# Autodesk Inventor assembly: rotor-housing-assembly
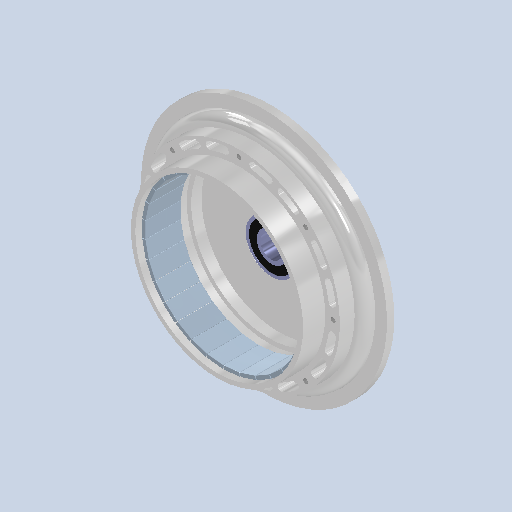
[picture p0: Inventor's stored thumbnail of the model, 512x512]
Saved by Autodesk Inventor 2022 (Build 260153000, 153)
## iProperties
Created: 2025-01-12
Part Number: rotor-housing-assembly
Document SubType Name: Assembly
Designer: Home
Author: Home
## Documents named in this file (4)
- D:\YandexDisk\Voltbro\xSets\components\HubWheel-10\rotor-housing-assembly.iam
- D:\YandexDisk\Voltbro\xSets\components\HubWheel-10\rotor-disc.ipt
- D:\YandexDisk\Voltbro\xSets\components\HubWheel-10\magnet_11x24-x2_5.ipt
- D:\YandexDisk\Voltbro\xSets\components\HubWheel-10\components\bearings\6202-2rs_15x35x11.ipt
## Components (32 placed, 3 different names)
1. rotor-disc:1 — Mate:4, Tangent:1, Tangent:2, Flush:1, Insert:1
2. 6202-2rs_15x35x11:1 — Insert:1
3. magnet_11x24-x2_5:1 — Mate:3, Tangent:1, Tangent:2, Flush:1
4. magnet_11x24-x2_5:2
5. magnet_11x24-x2_5:3
6. magnet_11x24-x2_5:4
7. magnet_11x24-x2_5:5
8. magnet_11x24-x2_5:6
9. magnet_11x24-x2_5:7
10. magnet_11x24-x2_5:8
11. magnet_11x24-x2_5:9
12. magnet_11x24-x2_5:10
13. magnet_11x24-x2_5:11
14. magnet_11x24-x2_5:12
15. magnet_11x24-x2_5:13
16. magnet_11x24-x2_5:14
17. magnet_11x24-x2_5:15
18. magnet_11x24-x2_5:16
19. magnet_11x24-x2_5:17
20. magnet_11x24-x2_5:18
21. magnet_11x24-x2_5:19
22. magnet_11x24-x2_5:20
23. magnet_11x24-x2_5:21
24. magnet_11x24-x2_5:22
25. magnet_11x24-x2_5:23
26. magnet_11x24-x2_5:24
27. magnet_11x24-x2_5:25
28. magnet_11x24-x2_5:26
29. magnet_11x24-x2_5:27
30. magnet_11x24-x2_5:28
31. magnet_11x24-x2_5:29
32. magnet_11x24-x2_5:30
## Component patterns: (30 elements, first: magnet_11x24-x2_5:1)
## Relationships (6: Mate 2, Tangent 2, Flush 1, Insert 1)
- Mate:3 (-5.5 mm): magnet_11x24-x2_5:1
- Mate:4: rotor-disc:1
- Tangent:1: rotor-disc:1 ↔ magnet_11x24-x2_5:1
- Tangent:2: rotor-disc:1 ↔ magnet_11x24-x2_5:1
- Flush:1 (4.2 mm): rotor-disc:1 ↔ magnet_11x24-x2_5:1
- Insert:1: rotor-disc:1 ↔ 6202-2rs_15x35x11:1
